# Autodesk Inventor assembly: 240516_cup_final
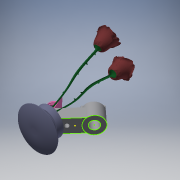
[picture p0: Inventor's stored thumbnail of the model, 180x180]
Saved by Autodesk Inventor 2016 (Build 200138000, 138)
## iProperties
Created: 2024-05-16
Part Number: 240516_cup_final
Material: 일반
Document SubType Name: Assembly
Designer: pc
Author: pc
## Documents named in this file (6)
- D:\CAD_HCH\240516\240516_cup_final.iam
- D:\CAD_HCH\240516\240516_cup.ipt
- D:\CAD_HCH\240516\240516_cup2.ipt
- D:\CAD_HCH\장미조립.iam
- D:\CAD_HCH\이름.ipt
- D:\CAD_HCH\240510\240510_3Dsketch06.ipt
## Components (6 placed, 5 different names)
1. 240516_cup:1 — 메이트:1
2. 240516_cup2:1 — 메이트:1
3. 장미조립:1 [sub-assembly]
4. 장미조립:2 [sub-assembly]
5. 이름:1
6. 240510_3Dsketch06:1
## Relationships (1: Mate 1)
- 메이트:1 [Mate]: 240516_cup:1 ↔ 240516_cup2:1
